# Autodesk Inventor assembly: DragBarLinkage2 Full
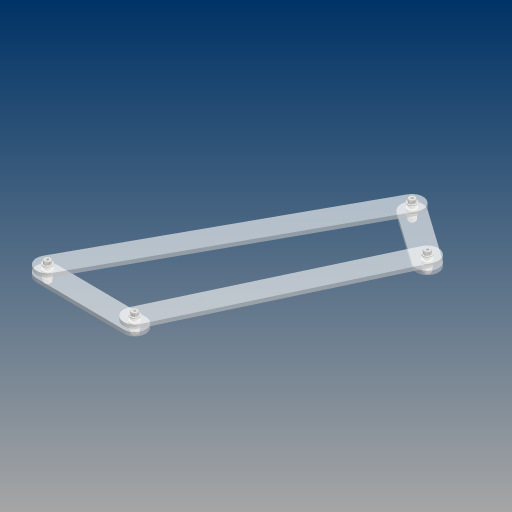
[picture p0: Inventor's stored thumbnail of the model, 512x512]
Saved by Autodesk Inventor 2024.3 (Build 283343000, 343)
## iProperties
Created: 2024-07-07
Part Number: DragBarLinkage2 Full
Document SubType Name: Assembly
Designer: Kenji
Sending System: Autodesk Inventor 2025
Preprocessor: ST-DEVELOPER v20
Title: DragBarLinkage2 Full.stp
Author: Kenji
## Documents named in this file (11)
- C:\Users\Kenji\Documents\FRC\Offseason 2024\DragBarLinkage2\DragBarLinkage2\DragBarLinkage2\DragBarLinkage2 Full.iam
- C:\Users\Kenji\Documents\FRC\Offseason 2024\DragBarLinkage2\DragLinkLinkage2 Bar1.ipt
- C:\Users\Kenji\Documents\FRC\Offseason 2024\DragBarLinkage2\DragLinkLinkage2 Bar2.ipt
- C:\Users\Kenji\Documents\FRC\Offseason 2024\DragBarLinkage2\DragLinkLinkage2 Bar3.ipt
- C:\Users\Kenji\Documents\FRC\Offseason 2024\DragBarLinkage2\6655K14_Thrust Ball Bearing.ipt
- C:\Users\Kenji\Documents\FRC\Offseason 2024\DragBarLinkage2\57155K306_Stainless Steel Ball Bearing.ipt
- C:\Users\Kenji\Documents\FRC\Offseason 2024\DragBarLinkage2\6655K14_Thrust Ball Bearing_1.ipt
- C:\Users\Kenji\Documents\FRC\Offseason 2024\DragBarLinkage2\DragBarLinkage2 Bar4.ipt
- C:\Users\Kenji\Documents\FRC\Offseason 2024\DragBarLinkage2\97135A414_High-Strength Steel Nylon-Insert Locknut.ipt
- C:\Users\Kenji\Documents\FRC\Offseason 2024\DragBarLinkage2\91259A581_Alloy Steel Shoulder Screw.ipt
- C:\Users\Kenji\Documents\FRC\Offseason 2024\DragBarLinkage2\92141A226_18-8 Stainless Steel Washer.ipt
## Components (28 placed, 9 different names)
1. DragLinkLinkage2 Bar1:1 — Mate:1, Mate:2, Mate:3, Mate:4, Mate:13, Mate:14, Mate:15, Mate:16
2. DragLinkLinkage2 Bar2:1 — Mate:5, Mate:6, Mate:7, Mate:8, Mate:18, Mate:19, Mate:20, Mate:21
3. DragLinkLinkage2 Bar3:1 — Mate:9, Mate:10, Mate:11, Mate:12, Mate:22, Mate:23, Mate:24, Mate:25
4. 6655K14_Thrust Ball Bearing:1 — Mate:13, Mate:14, Mate:18, Mate:19
5. 57155K306_Stainless Steel Ball Bearing:5 — Mate:5, Mate:7, Mate:55
6. 57155K306_Stainless Steel Ball Bearing:6 — Mate:9, Mate:11, Mate:40, Mate:41
7. 57155K306_Stainless Steel Ball Bearing:7 — Mate:6, Mate:8, Mate:49
8. 57155K306_Stainless Steel Ball Bearing:8 — Mate:1, Mate:4, Mate:38, Mate:39
9. 6655K14_Thrust Ball Bearing:2 — Mate:20, Mate:21, Mate:22, Mate:23
10. DragBarLinkage2 Bar4:1 — Mate:26, Mate:27, Mate:28, Mate:29, Mate:30, Mate:31
11. 6655K14_Thrust Ball Bearing:3 — Mate:15, Mate:16, Mate:17
12. 6655K14_Thrust Ball Bearing:4 — Mate:24, Mate:25, Mate:31
13. 57155K306_Stainless Steel Ball Bearing:9 — Mate:2, Mate:3, Mate:32, Mate:34
14. 57155K306_Stainless Steel Ball Bearing:10 — Mate:17, Mate:28, Mate:29, Mate:53
15. 57155K306_Stainless Steel Ball Bearing:11 — Mate:10, Mate:12, Mate:30, Mate:36, Mate:37
16. 57155K306_Stainless Steel Ball Bearing:12 — Mate:26, Mate:27, Mate:51
17. 97135A414_High-Strength Steel Nylon-Insert Locknut:1 — Mate:48, Mate:49
18. 97135A414_High-Strength Steel Nylon-Insert Locknut:2 — Mate:50, Mate:51
19. 97135A414_High-Strength Steel Nylon-Insert Locknut:3 — Mate:52, Mate:53
20. 97135A414_High-Strength Steel Nylon-Insert Locknut:4 — Mate:54, Mate:55
21. 91259A581_Alloy Steel Shoulder Screw:1 — Mate:32, Mate:33, Mate:35, Mate:52
22. 91259A581_Alloy Steel Shoulder Screw:2 — Mate:43, Mate:47, Mate:54
23. 91259A581_Alloy Steel Shoulder Screw:3 — Mate:42, Mate:46, Mate:50
24. 91259A581_Alloy Steel Shoulder Screw:4 — Mate:44, Mate:45, Mate:48
25. 92141A226_18-8 Stainless Steel Washer:1 — Mate:33, Mate:34, Mate:35
26. 92141A226_18-8 Stainless Steel Washer:2 — Mate:38, Mate:39, Mate:43, Mate:47
27. 92141A226_18-8 Stainless Steel Washer:3 — Mate:40, Mate:41, Mate:44, Mate:45
28. 92141A226_18-8 Stainless Steel Washer:4 — Mate:36, Mate:37, Mate:42, Mate:46
## Relationships (55: Mate 55)
- Mate:1: DragLinkLinkage2 Bar1:1 ↔ 57155K306_Stainless Steel Ball Bearing:8
- Mate:2: DragLinkLinkage2 Bar1:1 ↔ 57155K306_Stainless Steel Ball Bearing:9
- Mate:3: DragLinkLinkage2 Bar1:1 ↔ 57155K306_Stainless Steel Ball Bearing:9
- Mate:4: DragLinkLinkage2 Bar1:1 ↔ 57155K306_Stainless Steel Ball Bearing:8
- Mate:5: DragLinkLinkage2 Bar2:1 ↔ 57155K306_Stainless Steel Ball Bearing:5
- Mate:6: DragLinkLinkage2 Bar2:1 ↔ 57155K306_Stainless Steel Ball Bearing:7
- Mate:7: DragLinkLinkage2 Bar2:1 ↔ 57155K306_Stainless Steel Ball Bearing:5
- Mate:8: DragLinkLinkage2 Bar2:1 ↔ 57155K306_Stainless Steel Ball Bearing:7
- Mate:9: DragLinkLinkage2 Bar3:1 ↔ 57155K306_Stainless Steel Ball Bearing:6
- Mate:10: DragLinkLinkage2 Bar3:1 ↔ 57155K306_Stainless Steel Ball Bearing:11
- Mate:11: DragLinkLinkage2 Bar3:1 ↔ 57155K306_Stainless Steel Ball Bearing:6
- Mate:12: DragLinkLinkage2 Bar3:1 ↔ 57155K306_Stainless Steel Ball Bearing:11
- Mate:13: DragLinkLinkage2 Bar1:1 ↔ 6655K14_Thrust Ball Bearing:1
- Mate:14: DragLinkLinkage2 Bar1:1 ↔ 6655K14_Thrust Ball Bearing:1
- Mate:15: DragLinkLinkage2 Bar1:1 ↔ 6655K14_Thrust Ball Bearing:3
- Mate:16: DragLinkLinkage2 Bar1:1 ↔ 6655K14_Thrust Ball Bearing:3
- Mate:17: 6655K14_Thrust Ball Bearing:3 ↔ 57155K306_Stainless Steel Ball Bearing:10
- Mate:18: DragLinkLinkage2 Bar2:1 ↔ 6655K14_Thrust Ball Bearing:1
- Mate:19: DragLinkLinkage2 Bar2:1 ↔ 6655K14_Thrust Ball Bearing:1
- Mate:20: DragLinkLinkage2 Bar2:1 ↔ 6655K14_Thrust Ball Bearing:2
- Mate:21: DragLinkLinkage2 Bar2:1 ↔ 6655K14_Thrust Ball Bearing:2
- Mate:22: DragLinkLinkage2 Bar3:1 ↔ 6655K14_Thrust Ball Bearing:2
- Mate:23: DragLinkLinkage2 Bar3:1 ↔ 6655K14_Thrust Ball Bearing:2
- Mate:24: DragLinkLinkage2 Bar3:1 ↔ 6655K14_Thrust Ball Bearing:4
- Mate:25: DragLinkLinkage2 Bar3:1 ↔ 6655K14_Thrust Ball Bearing:4
- Mate:26: DragBarLinkage2 Bar4:1 ↔ 57155K306_Stainless Steel Ball Bearing:12
- Mate:27: DragBarLinkage2 Bar4:1 ↔ 57155K306_Stainless Steel Ball Bearing:12
- Mate:28: DragBarLinkage2 Bar4:1 ↔ 57155K306_Stainless Steel Ball Bearing:10
- Mate:29: DragBarLinkage2 Bar4:1 ↔ 57155K306_Stainless Steel Ball Bearing:10
- Mate:30: DragBarLinkage2 Bar4:1 ↔ 57155K306_Stainless Steel Ball Bearing:11
- Mate:31: DragBarLinkage2 Bar4:1 ↔ 6655K14_Thrust Ball Bearing:4
- Mate:32: 57155K306_Stainless Steel Ball Bearing:9 ↔ 91259A581_Alloy Steel Shoulder Screw:1
- Mate:33: 91259A581_Alloy Steel Shoulder Screw:1 ↔ 92141A226_18-8 Stainless Steel Washer:1
- Mate:34: 57155K306_Stainless Steel Ball Bearing:9 ↔ 92141A226_18-8 Stainless Steel Washer:1
- Mate:35: 91259A581_Alloy Steel Shoulder Screw:1 ↔ 92141A226_18-8 Stainless Steel Washer:1
- Mate:36: 57155K306_Stainless Steel Ball Bearing:11 ↔ 92141A226_18-8 Stainless Steel Washer:4
- Mate:37: 57155K306_Stainless Steel Ball Bearing:11 ↔ 92141A226_18-8 Stainless Steel Washer:4
- Mate:38: 57155K306_Stainless Steel Ball Bearing:8 ↔ 92141A226_18-8 Stainless Steel Washer:2
- Mate:39: 57155K306_Stainless Steel Ball Bearing:8 ↔ 92141A226_18-8 Stainless Steel Washer:2
- Mate:40: 57155K306_Stainless Steel Ball Bearing:6 ↔ 92141A226_18-8 Stainless Steel Washer:3
- Mate:41: 57155K306_Stainless Steel Ball Bearing:6 ↔ 92141A226_18-8 Stainless Steel Washer:3
- Mate:42: 91259A581_Alloy Steel Shoulder Screw:3 ↔ 92141A226_18-8 Stainless Steel Washer:4
- Mate:43: 91259A581_Alloy Steel Shoulder Screw:2 ↔ 92141A226_18-8 Stainless Steel Washer:2
- Mate:44: 91259A581_Alloy Steel Shoulder Screw:4 ↔ 92141A226_18-8 Stainless Steel Washer:3
- Mate:45: 91259A581_Alloy Steel Shoulder Screw:4 ↔ 92141A226_18-8 Stainless Steel Washer:3
- Mate:46: 91259A581_Alloy Steel Shoulder Screw:3 ↔ 92141A226_18-8 Stainless Steel Washer:4
- Mate:47: 91259A581_Alloy Steel Shoulder Screw:2 ↔ 92141A226_18-8 Stainless Steel Washer:2
- Mate:48: 97135A414_High-Strength Steel Nylon-Insert Locknut:1 ↔ 91259A581_Alloy Steel Shoulder Screw:4
- Mate:49: 57155K306_Stainless Steel Ball Bearing:7 ↔ 97135A414_High-Strength Steel Nylon-Insert Locknut:1
- Mate:50: 97135A414_High-Strength Steel Nylon-Insert Locknut:2 ↔ 91259A581_Alloy Steel Shoulder Screw:3
- Mate:51: 57155K306_Stainless Steel Ball Bearing:12 ↔ 97135A414_High-Strength Steel Nylon-Insert Locknut:2
- Mate:52: 97135A414_High-Strength Steel Nylon-Insert Locknut:3 ↔ 91259A581_Alloy Steel Shoulder Screw:1
- Mate:53: 57155K306_Stainless Steel Ball Bearing:10 ↔ 97135A414_High-Strength Steel Nylon-Insert Locknut:3
- Mate:54: 97135A414_High-Strength Steel Nylon-Insert Locknut:4 ↔ 91259A581_Alloy Steel Shoulder Screw:2
- Mate:55: 57155K306_Stainless Steel Ball Bearing:5 ↔ 97135A414_High-Strength Steel Nylon-Insert Locknut:4
